# Autodesk Inventor assembly: Робот RRO 2021
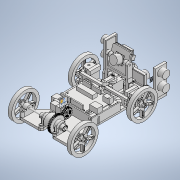
[picture p0: Inventor's stored thumbnail of the model, 180x180]
Saved by Autodesk Inventor 2020 (Build 240168000, 168)
## iProperties
Created: 2021-02-28
Part Number: Робот RRO 2021
Document SubType Name: Assembly
Designer: Антон
Author: Антон
## Documents named in this file (46)
- D:\Project\Robots\RRO 2021\Робот RRO 2021.iam
- D:\Project\Robots\RRO 2021\Body\Основа робота.ipt
- D:\Project\Robots\RRO 2021\Components\Кронштейн для двигателей серии N.ipt
- D:\Project\Robots\RRO 2021\Components\Servo SG90.ipt
- D:\Project\Robots\RRO 2021\Body\Основа рулевого механизма.ipt
- D:\Project\Robots\RRO 2021\Components\Подшипники\Подшипник 3 8 3.ipt
- D:\Project\Robots\RRO 2021\Components\Оси\Ось 3мм рулевого управления.ipt
- D:\Project\Robots\RRO 2021\Body\Деталь крепления диска к поворотному механизму.ipt
- D:\Project\Robots\RRO 2021\Components\Оси\Ось 3мм колеса.ipt
- D:\Project\Robots\RRO 2021\Components\Колесо D60 под ось моторов серии N.ipt
- D:\Project\Robots\RRO 2021\Body\Втулка между подшипниками рулевого управления.ipt
- D:\Project\Robots\RRO 2021\Components\Оси\Ось балки рулевого управления ведущая.ipt
- D:\Project\Robots\RRO 2021\Body\Балка рулевого управления ведущая.ipt
- D:\Project\Robots\RRO 2021\Body\Деталь крепления диска к поворотному механизму_ЗЕРКАЛО1.ipt
- D:\Project\Robots\RRO 2021\Body\Стойка под электроннику.ipt
- D:\Project\Robots\RRO 2021\Components\Arduino UNO.ipt
- D:\Project\Robots\RRO 2021\Body\Крепление камеры.ipt
- D:\Project\Robots\RRO 2021\Components\nVision lipo battery.ipt
- D:\Project\Robots\RRO 2021\Components\Micro Gearmotors.ipt
- D:\Project\Robots\RRO 2021\Components\Trackingcam (Applied robotics).ipt
- D:\Project\Robots\RRO 2021\Body\Стойка для камеры.ipt
- D:\Project\Robots\RRO 2021\Components\Подшипники\Подшипник 2 5 2,5.ipt
- D:\Project\Robots\RRO 2021\Components\Оси\Ось 2мм рулевой сервы.ipt
- D:\Project\Robots\RRO 2021\Body\Поворотный рычаг для сервы.ipt
- D:\Project\Robots\RRO 2021\Body\Крепление камеры к корпусу.ipt
- D:\Project\Robots\RRO 2021\Body\Крепление камеры к корпусу_ЗЕРКАЛО.ipt
- D:\Project\Robots\RRO 2021\Body\Поворотный стоппер.ipt
- D:\Project\Robots\RRO 2021\Body\Крышка стойки подшипника 3мм.ipt
- D:\Project\Robots\RRO 2021\Body\Стойки камеры.ipt
- D:\Project\Robots\RRO 2021\Body\Съемная стойка сервы.ipt
- D:\Project\Robots\RRO 2021\Body\Поворотный стоппер_ЗЕРКАЛО.ipt
- D:\Project\Robots\RRO 2021\Body\Крышка поворотного кулака.ipt
- D:\Project\Robots\RRO 2021\Components\Ultrasonic HC-SRO4.ipt
- D:\Project\Robots\RRO 2021\Body\Крышка аккумулятора.ipt
- D:\Project\Robots\RRO 2021\Body\Стойка подшипника 3мм.ipt
- D:\Project\Robots\RRO 2021\Components\Оси\Ось 3мм задняя.ipt
- D:\Project\Robots\RRO 2021\Body\Крепление ультрасоника.ipt
- D:\Project\Robots\RRO 2021\Body\Крепление ультрасоника вертикальная.ipt
- D:\Project\Robots\RRO 2021\Body\Крепление ультрасоника вертикальная_ЗЕРКАЛО.ipt
- D:\Project\Robots\RRO 2021\Components\Дифференциал.ipt
- D:\Project\Robots\RRO 2021\Body\Ведущая шестерня дифференециала.ipt
- D:\Project\Robots\RRO 2021\Components\Подшипники\Подшипник 10 15 4.ipt
- D:\Project\Robots\RRO 2021\Body\Крепление дифференциала.ipt
- D:\Project\Robots\RRO 2021\Body\Переходник с дифференциала на ось 3мм.ipt
- D:\Project\Robots\RRO 2021\Body\Крепление двигателя.ipt
- D:\Project\Robots\RRO 2021\Components\Оси\Ось мотора серии N.ipt
## Components (76 placed, 45 different names)
1. Основа робота:1 — Жесткий:130, Жесткий:135, Жесткий:138, Жесткий:140, Жесткий:143, Жесткий:145, Жесткий:152, Жесткий:153, Жесткий:161, Жесткий:162, Жесткий:168
2. Стойки камеры:1 — Жесткий:98
3. Стойки камеры:2 — Жесткий:95, Жесткий:99
4. Стойки камеры:3 — Жесткий:97
5. Стойки камеры:4 — Жесткий:96
6. Trackingcam (Applied robotics):1 — Жесткий:95, Жесткий:96, Жесткий:97, Жесткий:98
7. Крепление камеры:1 — С поворотом:32, Жесткий:99
8. Стойка для камеры:1 — С поворотом:32, Жесткий:106, Жесткий:107
9. Крепление камеры к корпусу_ЗЕРКАЛО:1 — Жесткий:106, Жесткий:130
10. Крепление камеры к корпусу:1 — Жесткий:107
11. Основа рулевого механизма:1 — Жесткий:45, Жесткий:46, Жесткий:100, Жесткий:101, Жесткий:102, Жесткий:103, Жесткий:135
12. Съемная стойка сервы:1 — Жесткий:101
13. Servo SG90:2 — С поворотом:26, Жесткий:100
14. Поворотный рычаг для сервы:1 — С поворотом:26, Жесткий:149
15. Подшипник 2*5*2.5:2 — С поворотом:25, Жесткий:149
16. Ось 2мм рулевой сервы:1 — С поворотом:24, С поворотом:25
17. Подшипник 2*5*2.5:1 — С поворотом:24, Жесткий:173
18. Балка рулевого управления:1 — С поворотом:35, С поворотом:36, Жесткий:173
19. Поворотный стоппер:2 — Жесткий:102
20. Поворотный стоппер_ЗЕРКАЛО:1 — Жесткий:103
21. Крышка аккумулятора:1 — Жесткий:108
22. nVision lipo battery:1 — Жесткий:54
23. Стойка под электроннику:1 — Жесткий:53, Жесткий:54, Жесткий:108, Жесткий:140
24. Arduino UNO:1 — Жесткий:53
25. Ось 3мм задняя:2 — Жесткий:118, Жесткий:165
26. Переходник с дифференциала на ось 3мм:1 — Жесткий:165, Жесткий:171
27. Дифференциал:1 — С поворотом:158, Жесткий:166, ЗубчПер:1, Жесткий:171
28. Переходник с дифференциала на ось 3мм:2 — Жесткий:166, Жесткий:170
29. Ось 3мм задняя:1 — Жесткий:119, Жесткий:170
30. Крепление ультрасоника вертикальная_ЗЕРКАЛО:1 — Жесткий:143, Жесткий:148
31. Ultrasonic HC-SRO4:3 — Жесткий:148
32. Ultrasonic HC-SRO4:1 — Жесткий:146
33. Крепление ультрасоника горизонтальное:1 — Жесткий:138, Жесткий:146
34. Крепление ультрасоника вертикальное:1 — Жесткий:145, Жесткий:147
35. Ultrasonic HC-SRO4:2 — Жесткий:147
36. Крышка поворотного кулака:2 — Жесткий:137
37. Деталь крепления диска к поворотному механизму:1 — Жесткий:13, Жесткий:14, Жесткий:34, Жесткий:125, Жесткий:137
38. Втулка между подшипниками рулевого управления:1 — Жесткий:11, Жесткий:12
39. Крышка поворотного кулака:1 — Жесткий:136
40. Деталь крепления диска к поворотному механизму_ЗЕРКАЛО1:1 — Жесткий:37, Жесткий:38, Жесткий:39, Жесткий:44, Жесткий:136
41. Втулка между подшипниками рулевого управления:2
42. Крепление двигателя:1 — Жесткий:168, Жесткий:172
43. Кронштейн для двигателей серии N:1 — Жесткий:172, Жесткий:174
44. Micro Gearmotors:1 — С поворотом:160, Жесткий:174
45. Ось мотора серии N:1 — Жесткий:169, С поворотом:160
46. Ведущая шестерня дифференециала:1 — Жесткий:169, ЗубчПер:1
47. Крышка стойки подшипника 3мм:1 — Жесткий:109, Жесткий:110
48. Подшипник 3*8*3:9 — Жесткий:109
49. Стойка подшипника 3мм:1 — Жесткий:110, Жесткий:153
50. Крепление дифференциала:2 — Жесткий:160, Жесткий:162
51. Подшипник 10 15 4:1 — С поворотом:158, Жесткий:160
52. Крепление дифференциала:1 — Жесткий:159, Жесткий:161
53. Подшипник 10 15 4:2 — Жесткий:159
54. Крышка стойки подшипника 3мм:4 — Жесткий:114, Жесткий:163
55. Подшипник 3*8*3:10 — Жесткий:163
56. Стойка подшипника 3мм:4 — Жесткий:114, Жесткий:152
57. Колесо D60 под ось моторов серии N:1:1 — Жесткий:9
58. Колесо D60 под ось моторов серии N:1:2
59. Колесо D60 под ось моторов серии N:1:4 — Жесткий:118
60. Колесо D60 под ось моторов серии N:1:3 — Жесткий:119
61. Ось 3мм рулевого управления:3 — С поворотом:14, Жесткий:14
62. Ось 3мм колеса:1 — Жесткий:9, С поворотом:12
63. Ось 3мм рулевого управления:1 — С поворотом:13, Жесткий:13
64. Ось балки рулевого управления ведущая:2 — Жесткий:34, С поворотом:35
65. Подшипник 3*8*3:1 — Жесткий:12
66. Подшипник 3*8*3:2 — С поворотом:13, Жесткий:45
67. Подшипник 3*8*3:3 — С поворотом:14
68. Подшипник 3*8*3:4 — Жесткий:11, С поворотом:12, Жесткий:125
69. Ось 3мм колеса:2
70. Ось 3мм рулевого управления:4 — С поворотом:16, Жесткий:44
71. Ось балки рулевого управления ведущая:1 — Жесткий:39, С поворотом:36
72. Ось 3мм рулевого управления:5 — Жесткий:37
73. Подшипник 3*8*3:7
74. Подшипник 3*8*3:8 — Жесткий:38
75. Подшипник 3*8*3:6 — С поворотом:16, Жесткий:46
76. Подшипник 3*8*3:5
## Relationships (78: WeldJoint 63, RevoluteJoint 14, RelateRotation 1)
- Жесткий:9 [WeldJoint]: Колесо D60 под ось моторов серии N:1:1 ↔ Ось 3мм колеса:1
- Жесткий:11 [WeldJoint]: Втулка между подшипниками рулевого управления:1 ↔ Подшипник 3*8*3:4
- Жесткий:12 [WeldJoint]: Втулка между подшипниками рулевого управления:1 ↔ Подшипник 3*8*3:1
- С поворотом:12 [RevoluteJoint]: Ось 3мм колеса:1 ↔ Подшипник 3*8*3:4
- С поворотом:13 [RevoluteJoint]: Ось 3мм рулевого управления:1 ↔ Подшипник 3*8*3:2
- С поворотом:14 [RevoluteJoint]: Ось 3мм рулевого управления:3 ↔ Подшипник 3*8*3:3
- Жесткий:13 [WeldJoint]: Деталь крепления диска к поворотному механизму:1 ↔ Ось 3мм рулевого управления:1
- Жесткий:14 [WeldJoint]: Деталь крепления диска к поворотному механизму:1 ↔ Ось 3мм рулевого управления:3
- [WeldJoint]: Колесо D60 под ось моторов серии N:1:2 ↔ Ось 3мм колеса:2
- [WeldJoint]: Втулка между подшипниками рулевого управления:2 ↔ Подшипник 3*8*3:8
- [WeldJoint]: Втулка между подшипниками рулевого управления:2 ↔ Подшипник 3*8*3:5
- [RevoluteJoint]: Ось 3мм колеса:2 ↔ Подшипник 3*8*3:8
- С поворотом:16 [RevoluteJoint]: Ось 3мм рулевого управления:4 ↔ Подшипник 3*8*3:6
- [RevoluteJoint]: Ось 3мм рулевого управления:5 ↔ Подшипник 3*8*3:7
- Жесткий:34 [WeldJoint]: Деталь крепления диска к поворотному механизму:1 ↔ Ось балки рулевого управления ведущая:2
- Жесткий:37 [WeldJoint]: Деталь крепления диска к поворотному механизму_ЗЕРКАЛО1:1 ↔ Ось 3мм рулевого управления:5
- Жесткий:38 [WeldJoint]: Деталь крепления диска к поворотному механизму_ЗЕРКАЛО1:1 ↔ Подшипник 3*8*3:8
- Жесткий:39 [WeldJoint]: Деталь крепления диска к поворотному механизму_ЗЕРКАЛО1:1 ↔ Ось балки рулевого управления ведущая:1
- Жесткий:44 [WeldJoint]: Деталь крепления диска к поворотному механизму_ЗЕРКАЛО1:1 ↔ Ось 3мм рулевого управления:4
- Жесткий:45 [WeldJoint]: Основа рулевого механизма:1 ↔ Подшипник 3*8*3:2
- Жесткий:46 [WeldJoint]: Основа рулевого механизма:1 ↔ Подшипник 3*8*3:6
- Жесткий:53 [WeldJoint]: Стойка под электроннику:1 ↔ Arduino UNO:1
- Жесткий:54 [WeldJoint]: nVision lipo battery:1 ↔ Стойка под электроннику:1
- С поворотом:24 [RevoluteJoint]: Ось 2мм рулевой сервы:1 ↔ Подшипник 2*5*2.5:1
- С поворотом:25 [RevoluteJoint]: Подшипник 2*5*2.5:2 ↔ Ось 2мм рулевой сервы:1
- С поворотом:26 [RevoluteJoint]: Servo SG90:2 ↔ Поворотный рычаг для сервы:1
- С поворотом:32 [RevoluteJoint] (-0.15 mm): Крепление камеры:1 ↔ Стойка для камеры:1
- Жесткий:95 [WeldJoint]: Стойки камеры:2 ↔ Trackingcam (Applied robotics):1
- Жесткий:96 [WeldJoint]: Стойки камеры:4 ↔ Trackingcam (Applied robotics):1
- Жесткий:97 [WeldJoint]: Стойки камеры:3 ↔ Trackingcam (Applied robotics):1
- Жесткий:98 [WeldJoint]: Стойки камеры:1 ↔ Trackingcam (Applied robotics):1
- Жесткий:99 [WeldJoint]: Стойки камеры:2 ↔ Крепление камеры:1
- Жесткий:100 [WeldJoint]: Основа рулевого механизма:1 ↔ Servo SG90:2
- Жесткий:101 [WeldJoint]: Основа рулевого механизма:1 ↔ Съемная стойка сервы:1
- Жесткий:102 [WeldJoint] (0.05 mm): Основа рулевого механизма:1 ↔ Поворотный стоппер:2
- Жесткий:103 [WeldJoint] (0.05 mm): Основа рулевого механизма:1 ↔ Поворотный стоппер_ЗЕРКАЛО:1
- Жесткий:106 [WeldJoint] (-0.1 mm): Стойка для камеры:1 ↔ Крепление камеры к корпусу_ЗЕРКАЛО:1
- Жесткий:107 [WeldJoint] (-0.1 mm): Стойка для камеры:1 ↔ Крепление камеры к корпусу:1
- Жесткий:108 [WeldJoint]: Крышка аккумулятора:1 ↔ Стойка под электроннику:1
- Жесткий:109 [WeldJoint] (-0.05 mm): Крышка стойки подшипника 3мм:1 ↔ Подшипник 3*8*3:9
- Жесткий:110 [WeldJoint]: Крышка стойки подшипника 3мм:1 ↔ Стойка подшипника 3мм:1
- Жесткий:114 [WeldJoint]: Крышка стойки подшипника 3мм:4 ↔ Стойка подшипника 3мм:4
- Жесткий:118 [WeldJoint]: Ось 3мм задняя:2 ↔ Колесо D60 под ось моторов серии N:1:4
- Жесткий:119 [WeldJoint]: Ось 3мм задняя:1 ↔ Колесо D60 под ось моторов серии N:1:3
- Жесткий:125 [WeldJoint]: Деталь крепления диска к поворотному механизму:1 ↔ Подшипник 3*8*3:4
- С поворотом:35 [RevoluteJoint]: Балка рулевого управления:1 ↔ Ось балки рулевого управления ведущая:2
- С поворотом:36 [RevoluteJoint]: Балка рулевого управления:1 ↔ Ось балки рулевого управления ведущая:1
- Жесткий:130 [WeldJoint]: Основа робота:1 ↔ Крепление камеры к корпусу_ЗЕРКАЛО:1
- Жесткий:135 [WeldJoint]: Основа робота:1 ↔ Основа рулевого механизма:1
- Жесткий:136 [WeldJoint]: Крышка поворотного кулака:1 ↔ Деталь крепления диска к поворотному механизму_ЗЕРКАЛО1:1
- Жесткий:137 [WeldJoint]: Крышка поворотного кулака:2 ↔ Деталь крепления диска к поворотному механизму:1
- Жесткий:138 [WeldJoint]: Основа робота:1 ↔ Крепление ультрасоника горизонтальное:1
- Жесткий:140 [WeldJoint]: Основа робота:1 ↔ Стойка под электроннику:1
- Жесткий:143 [WeldJoint]: Основа робота:1 ↔ Крепление ультрасоника вертикальная_ЗЕРКАЛО:1
- Жесткий:145 [WeldJoint]: Основа робота:1 ↔ Крепление ультрасоника вертикальное:1
- Жесткий:146 [WeldJoint]: Ultrasonic HC-SRO4:1 ↔ Крепление ультрасоника горизонтальное:1
- Жесткий:147 [WeldJoint]: Крепление ультрасоника вертикальное:1 ↔ Ultrasonic HC-SRO4:2
- Жесткий:148 [WeldJoint]: Крепление ультрасоника вертикальная_ЗЕРКАЛО:1 ↔ Ultrasonic HC-SRO4:3
- Жесткий:149 [WeldJoint]: Поворотный рычаг для сервы:1 ↔ Подшипник 2*5*2.5:2
- Жесткий:152 [WeldJoint]: Основа робота:1 ↔ Стойка подшипника 3мм:4
- Жесткий:153 [WeldJoint]: Основа робота:1 ↔ Стойка подшипника 3мм:1
- С поворотом:158 [RevoluteJoint]: Дифференциал:1 ↔ Подшипник 10 15 4:1
- Жесткий:159 [WeldJoint]: Крепление дифференциала:1 ↔ Подшипник 10 15 4:2
- Жесткий:160 [WeldJoint]: Крепление дифференциала:2 ↔ Подшипник 10 15 4:1
- Жесткий:161 [WeldJoint]: Основа робота:1 ↔ Крепление дифференциала:1
- Жесткий:162 [WeldJoint]: Основа робота:1 ↔ Крепление дифференциала:2
- Жесткий:163 [WeldJoint] (-0.05 mm): Крышка стойки подшипника 3мм:4 ↔ Подшипник 3*8*3:10
- Жесткий:165 [WeldJoint]: Ось 3мм задняя:2 ↔ Переходник с дифференциала на ось 3мм:1
- Жесткий:166 [WeldJoint]: Дифференциал:1 ↔ Переходник с дифференциала на ось 3мм:2
- Жесткий:170 [WeldJoint]: Переходник с дифференциала на ось 3мм:2 ↔ Ось 3мм задняя:1
- Жесткий:168 [WeldJoint]: Основа робота:1 ↔ Крепление двигателя:1
- Жесткий:169 [WeldJoint]: Ось мотора серии N:1 ↔ Ведущая шестерня дифференециала:1
- ЗубчПер:1 [RelateRotation] (2 ul): Дифференциал:1 ↔ Ведущая шестерня дифференециала:1
- С поворотом:160 [RevoluteJoint]: Micro Gearmotors:1 ↔ Ось мотора серии N:1
- Жесткий:171 [WeldJoint]: Переходник с дифференциала на ось 3мм:1 ↔ Дифференциал:1
- Жесткий:172 [WeldJoint]: Крепление двигателя:1 ↔ Кронштейн для двигателей серии N:1
- Жесткий:173 [WeldJoint]: Подшипник 2*5*2.5:1 ↔ Балка рулевого управления:1
- Жесткий:174 [WeldJoint]: Кронштейн для двигателей серии N:1 ↔ Micro Gearmotors:1
## Named parameters: d71_d54 = 0 mm, d72_d55 = 180 deg, d73_d56 = 0 mm, d74_d57 = -3.272221 deg, d75_d60 = 180 deg, d76_d61 = 0 deg, d77_d42 = 0 mm, d79_d47 = 0 mm, d80_d48 = 0 mm, d81_d49 = 0 mm, d82_d50 = 0 deg
